# Autodesk Inventor assembly: Sestava_kryt_na_displej_PCB
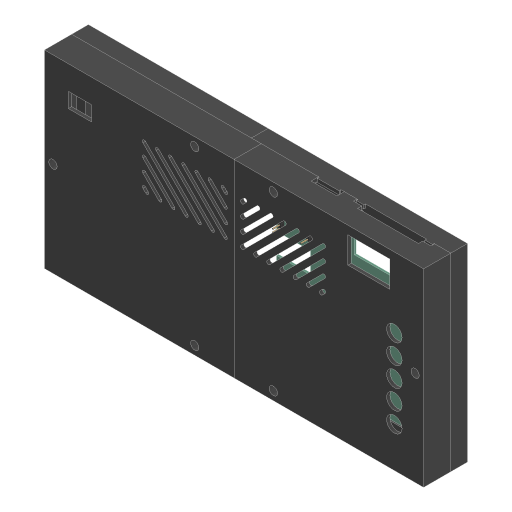
[picture p0: Inventor's stored thumbnail of the model, 512x512]
Saved by Autodesk Inventor 2023 (Build 270158000, 158)
## iProperties
Created: 2024-12-11
Part Number: Sestava_kryt_na_displej_PCB
Document SubType Name: Assembly
Designer: Marek
Author: Marek
## Documents named in this file (6)
- C:\Users\Marek\Documents\Inventor\displej\Sestava_kryt_na_displej_PCB.iam
- C:\Users\Marek\Documents\Inventor\displej\display_cover_part1.ipt
- C:\Users\Marek\Documents\Inventor\displej\pcb\displej_pcb.iam
- C:\Users\Marek\Documents\Inventor\displej\display_cover_part2.ipt
- C:\Users\Marek\Documents\Inventor\displej\display_cover_part1_back.ipt
- C:\Users\Marek\Documents\Inventor\displej\display_cover_part2_back.ipt
## Components (5 placed, 5 different names)
1. display_cover_part1:1 — Proti sobě:2, Proti sobě:3, Proti sobě:4, Proti sobě:5, Stejný směr:1, Stejný směr:2, Proti sobě:7, Vložit:1
2. display_cover_part2:1 — Proti sobě:2, Proti sobě:3, Proti sobě:4, Proti sobě:6, Stejný směr:3, Stejný směr:4
3. display_cover_part1_back:1 — Proti sobě:5, Stejný směr:1, Stejný směr:2
4. display_cover_part2_back:1 — Proti sobě:6, Stejný směr:3, Stejný směr:4
5. displej_pcb:1 [sub-assembly] — Proti sobě:7, Vložit:1
## Relationships (11: Mate 6, Flush 4, Insert 1)
- Proti sobě:2 [Mate]: display_cover_part1:1 ↔ display_cover_part2:1
- Proti sobě:3 [Mate]: display_cover_part1:1 ↔ display_cover_part2:1
- Proti sobě:4 [Mate]: display_cover_part1:1 ↔ display_cover_part2:1
- Proti sobě:5 [Mate]: display_cover_part1:1 ↔ display_cover_part1_back:1
- Stejný směr:1 [Flush]: display_cover_part1:1 ↔ display_cover_part1_back:1
- Stejný směr:2 [Flush]: display_cover_part1:1 ↔ display_cover_part1_back:1
- Proti sobě:6 [Mate]: display_cover_part2:1 ↔ display_cover_part2_back:1
- Stejný směr:3 [Flush]: display_cover_part2:1 ↔ display_cover_part2_back:1
- Stejný směr:4 [Flush]: display_cover_part2:1 ↔ display_cover_part2_back:1
- Proti sobě:7 [Mate]: display_cover_part1:1 ↔ displej_pcb:1
- Vložit:1 [Insert]: display_cover_part1:1 ↔ displej_pcb:1
